# Autodesk Inventor assembly: Case-D
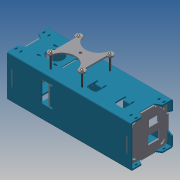
[picture p0: Inventor's stored thumbnail of the model, 180x180]
Saved by Autodesk Inventor 2017 (Build 210142000, 142)
## iProperties
Part Number: Case-D
Material: Genérico
Document SubType Name: Assembly
Designer: Leo
Author: Leo
## Documents named in this file (7)
- C:\Users\FABLAB\Documents\GitHub\actor-re-actor\models\inventor-caja\Case\Case-D.iam
- C:\Users\FABLAB\Documents\GitHub\actor-re-actor\models\inventor-caja\Case\Tapa Enchufes b.ipt
- C:\Users\FABLAB\Documents\GitHub\actor-re-actor\models\inventor-caja\Case\Carcasa.ipt
- C:\Users\FABLAB\Documents\GitHub\actor-re-actor\models\inventor-caja\Case\refuerzo interior B.ipt
- C:\Users\FABLAB\Documents\GitHub\actor-re-actor\models\inventor-caja\Case\tapa ventilador.ipt
- C:\Users\FABLAB\Documents\GitHub\actor-re-actor\models\inventor-caja\Case\protector carrete.ipt
- C:\Users\FABLAB\Documents\GitHub\actor-re-actor\models\inventor-caja\Case\Case-D\Design Accelerator\Conexión por perno1.iam
## Components (6 placed, 6 different names)
1. Carcasa:1 — Coincidencia:11, Nivelación:10, Nivelación:11, Nivelación:13, Nivelación:15, Coincidencia:3, Nivelación:17
2. Tapa Enchufes b:1 — Coincidencia:11, Nivelación:16, Nivelación:10
3. tapa ventilador:1 — Nivelación:11, Nivelación:12, Nivelación:13
4. refuerzo interior B:1 — Nivelación:14, Nivelación:15, Coincidencia:3
5. protector carrete:1 — Nivelación:17, Nivelación:18, Nivelación:19, Coincidencia:12, Coincidencia:13
6. Conexión por perno:1 [sub-assembly] — Coincidencia:12, Coincidencia:13
## Relationships (14: Flush 10, Mate 4)
- Coincidencia:11 [Mate]: Carcasa:1 ↔ Tapa Enchufes b:1
- Nivelación:16 [Flush]: Tapa Enchufes b:1
- Nivelación:10 [Flush]: Carcasa:1 ↔ Tapa Enchufes b:1
- Nivelación:11 [Flush]: Carcasa:1 ↔ tapa ventilador:1
- Nivelación:12 [Flush]: tapa ventilador:1
- Nivelación:13 [Flush]: Carcasa:1 ↔ tapa ventilador:1
- Nivelación:14 [Flush]: refuerzo interior B:1
- Nivelación:15 [Flush]: Carcasa:1 ↔ refuerzo interior B:1
- Coincidencia:3 [Mate]: Carcasa:1 ↔ refuerzo interior B:1
- Nivelación:17 [Flush] (38 mm): Carcasa:1 ↔ protector carrete:1
- Nivelación:18 [Flush]: protector carrete:1
- Nivelación:19 [Flush]: protector carrete:1
- Coincidencia:12 [Mate]: protector carrete:1 ↔ Conexión por perno:1
- Coincidencia:13 [Mate]: protector carrete:1 ↔ Conexión por perno:1
